# Autodesk Inventor assembly: mainstepper
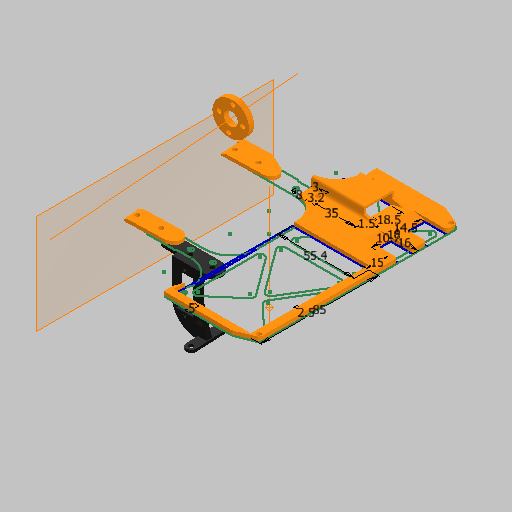
[picture p0: Inventor's stored thumbnail of the model, 512x512]
Saved by Autodesk Inventor 2026 (Build 300175000, 175)
## iProperties
Created: 2026-07-30
Part Number: mainstepper
Document SubType Name: Assembly
Designer: admin
Author: admin
## Documents named in this file (6)
- C:\Users\admin\Downloads\Bowling-ChinaRobotChalenge\3d-models\mainstepper.iam
- C:\Users\admin\Downloads\Bowling-ChinaRobotChalenge\3d-models\frame.ipt
- C:\Users\admin\Downloads\Bowling-ChinaRobotChalenge\3d-prints\servholder.ipt
- C:\Users\admin\Downloads\Bowling-ChinaRobotChalenge\3d-models\bldcholder.ipt
- C:\Users\admin\Downloads\Bowling-ChinaRobotChalenge\3d-models\ball.ipt
- C:\Users\admin\Downloads\Bowling-ChinaRobotChalenge\3d-models\vall.ipt
## Components (5 placed, 5 different names)
1. frame:1 — Совмещение:1, Заподлицо:2, Заподлицо:3, Заподлицо:4, Заподлицо:5, Совмещение:2, Совмещение:3, Заподлицо:6, Заподлицо:7, Заподлицо:9
2. servholder:1 — Заподлицо:2, Заподлицо:4, Заподлицо:9
3. bldcholder:1 — Заподлицо:3, Заподлицо:5, Совмещение:2, Совмещение:3, Совмещение:4
4. ball:1 — Заподлицо:6, Заподлицо:7
5. vall:1 — Заподлицо:8
## Relationships (13: Flush 8, Mate 4, Angle 1)
- Совмещение:1 [Mate]: frame:1
- Заподлицо:2 [Flush] (-9 mm): frame:1 ↔ servholder:1
- Заподлицо:3 [Flush]: frame:1 ↔ bldcholder:1
- Заподлицо:4 [Flush]: frame:1 ↔ servholder:1
- Заподлицо:5 [Flush]: frame:1 ↔ bldcholder:1
- Совмещение:2 [Mate]: frame:1 ↔ bldcholder:1
- Совмещение:3 [Mate]: frame:1 ↔ bldcholder:1
- Заподлицо:6 [Flush]: frame:1 ↔ ball:1
- Заподлицо:7 [Flush]: frame:1 ↔ ball:1
- Совмещение:4 [Mate]: bldcholder:1
- Угол:1 [Angle] (0 deg)
- Заподлицо:8 [Flush]: vall:1
- Заподлицо:9 [Flush]: frame:1 ↔ servholder:1
